# Autodesk Inventor assembly: Assembly_xiao_adapter
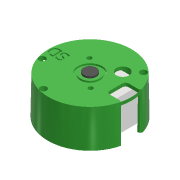
[picture p0: Inventor's stored thumbnail of the model, 180x180]
Saved by Autodesk Inventor 2022 (Build 260153000, 153)
## iProperties
Created: 2023-05-23
Part Number: Assembly_xiao_adapter
Document SubType Name: Assembly
Designer: diederichbenedict
Author: diederichbenedict
## Documents named in this file (5)
- C:\Users\diederichbenedict\Dropbox\Dokumente\Promotion\PROJECTS\Matchboxscope\INVENTOR\RELEASE\InjectionMolded\Assembly_xiao_adapter.iam
- C:\Users\diederichbenedict\Dropbox\Dokumente\Promotion\PROJECTS\Matchboxscope\INVENTOR\RELEASE\InjectionMolded\IM_Matchboxscope_base.ipt
- C:\Users\diederichbenedict\Dropbox\Dokumente\Promotion\PROJECTS\Matchboxscope\INVENTOR\RELEASE\InjectionMolded\00_Seeeduino Xiao.ipt
- C:\Users\diederichbenedict\Dropbox\Dokumente\Promotion\PROJECTS\Matchboxscope\INVENTOR\RELEASE\Matchboxscope\Workspace\00_ESP3-CAM.iam
- C:\Users\diederichbenedict\Dropbox\Dokumente\Promotion\PROJECTS\Matchboxscope\INVENTOR\RELEASE\InjectionMolded\IM_Matchboxscope_base_seeed_adapter.ipt
## Components (4 placed, 4 different names)
1. 00_Seeeduino Xiao:2 — Einfügen:2, Einfügen:3
2. 00_ESP3-CAM:1 [sub-assembly] — Einfügen:2, Fluchtend:1
3. IM_Matchboxscope_base_seeed_adapter:1 — Fluchtend:1
4. IM_Matchboxscope_base:1 — Einfügen:3
## Relationships (3: Insert 2, Flush 1)
- Einfügen:2 [Insert] (-2 mm): 00_Seeeduino Xiao:2 ↔ 00_ESP3-CAM:1
- Fluchtend:1 [Flush]: 00_ESP3-CAM:1 ↔ IM_Matchboxscope_base_seeed_adapter:1
- Einfügen:3 [Insert]: 00_Seeeduino Xiao:2 ↔ IM_Matchboxscope_base:1
